# Autodesk Inventor assembly: Solenoid Assembly
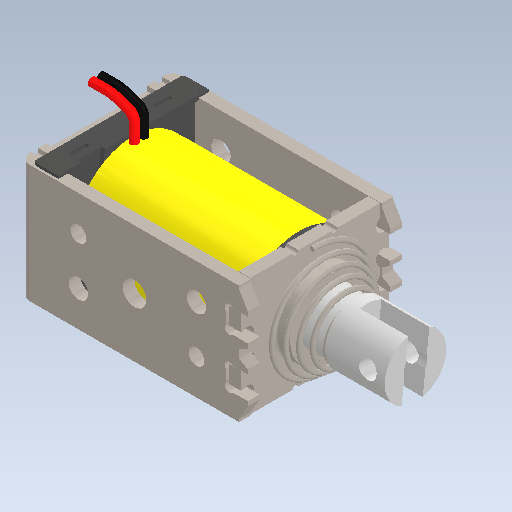
[picture p0: Inventor's stored thumbnail of the model, 512x512]
Saved by Autodesk Inventor 2020.3 (Build 243373010, 373A)
## iProperties
Created: 2019-10-22
Part Number: Solenoid Assembly
Document SubType Name: Assembly
Designer: Owner
Author: Owner
## Documents named in this file (3)
- D:\Designs\MK3PRO P1\E2\Solenoid Assembly.iam
- D:\Designs\MK3PRO P1\E2\SolenoidBody.ipt
- D:\Designs\MK3PRO P1\E2\SolenoidShaft.ipt
## Components (2 placed, 2 different names)
1. SolenoidBody:1 — Mate:1
2. SolenoidShaft:1 — Mate:1
## Relationships (1: Mate 1)
- Mate:1: SolenoidBody:1 ↔ SolenoidShaft:1
